# Autodesk Inventor assembly: sus1
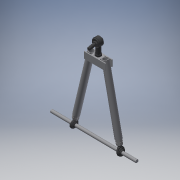
[picture p0: Inventor's stored thumbnail of the model, 180x180]
Saved by Autodesk Inventor 2018 (Build 220112000, 112)
## iProperties
Created: 2017-09-08
Part Number: sus1
Material: 一般
Document SubType Name: Assembly
Designer: mura5
Author: mura5
## Documents named in this file (8)
- C:\Users\mura5\Documents\RBBR\cart\Sus1.iam
- C:\Users\mura5\Documents\RBBR\cart\Rod1.iam
- C:\Users\mura5\Documents\RBBR\cart\Plate1.ipt
- C:\Users\mura5\Documents\RBBR\cart\Plate2.ipt
- C:\Users\mura5\Documents\RBBR\cart\iko_POS_14EC\AIS2016\POS 14ECBall.ipt
- C:\Users\mura5\Documents\RBBR\cart\Shaft14mm.ipt
- C:\Users\mura5\Documents\RBBR\cart\iko_LHSA_14\AIS2016\LHSA 14 Body1.ipt
- C:\Users\mura5\Documents\RBBR\cart\iko_LHSA_14\AIS2016\LHSA 14 Body2.ipt
## Components (10 placed, 7 different names)
1. POS 14ECBall:1 — 回転:1, 円柱状:1, ボール:4, メイト:9
2. Rod1:1 [sub-assembly] — 正接:2, 角度:1, メイト:2, ボール:4, メイト:6, メイト:7, 正接:3
3. Rod1:2 [sub-assembly] — ボール:2, 正接:1, 角度:2, メイト:3, メイト:5, メイト:8, 正接:4
4. Plate1:1 — 正接:1, 正接:2, フラッシュ:1, フラッシュ:2, メイト:1, フラッシュ:4, 正接:3, 正接:4
5. Plate2:1 — フラッシュ:1, フラッシュ:2, メイト:1, 角度:1, 角度:2, メイト:2, メイト:3, フラッシュ:3, メイト:4, リジッド:1, メイト:5, メイト:6, メイト:7, メイト:8
6. POS 14ECBall:2 — ボール:2, 回転:1, 円柱状:2, メイト:9
7. Shaft14mm:1 — 円柱状:1, 円柱状:2
8. Plate1:2 — フラッシュ:3, メイト:4, フラッシュ:4
9. LHSA 14 Body1:1 — リジッド:1, ボール:3
10. LHSA 14 Body2:1 — ボール:3
## Relationships (26: Mate 9, Tangent 4, Flush 4, BallJoint 3, CylindricalJoint 2, Angle 2, RevoluteJoint 1, WeldJoint 1)
- ボール:2 [BallJoint]: Rod1:2 ↔ POS 14ECBall:2
- 回転:1 [RevoluteJoint] (200 mm): POS 14ECBall:1 ↔ POS 14ECBall:2
- 円柱状:1 [CylindricalJoint]: POS 14ECBall:1 ↔ Shaft14mm:1
- 円柱状:2 [CylindricalJoint]: POS 14ECBall:2 ↔ Shaft14mm:1
- 正接:1 [Tangent]: Rod1:2 ↔ Plate1:1
- 正接:2 [Tangent]: Rod1:1 ↔ Plate1:1
- フラッシュ:1 [Flush] (-30 mm): Plate1:1 ↔ Plate2:1
- フラッシュ:2 [Flush]: Plate1:1 ↔ Plate2:1
- メイト:1 [Mate]: Plate1:1 ↔ Plate2:1
- 角度:1 [Angle] (-110 deg): Rod1:1 ↔ Plate2:1
- 角度:2 [Angle] (110 deg): Rod1:2 ↔ Plate2:1
- メイト:2 [Mate]: Rod1:1 ↔ Plate2:1
- メイト:3 [Mate]: Rod1:2 ↔ Plate2:1
- フラッシュ:3 [Flush]: Plate2:1 ↔ Plate1:2
- メイト:4 [Mate]: Plate2:1 ↔ Plate1:2
- フラッシュ:4 [Flush]: Plate1:1 ↔ Plate1:2
- リジッド:1 [WeldJoint]: Plate2:1 ↔ LHSA 14 Body1:1
- ボール:3 [BallJoint]: LHSA 14 Body1:1 ↔ LHSA 14 Body2:1
- ボール:4 [BallJoint]: POS 14ECBall:1 ↔ Rod1:1
- メイト:5 [Mate]: Rod1:2 ↔ Plate2:1
- メイト:6 [Mate]: Rod1:1 ↔ Plate2:1
- メイト:7 [Mate]: Rod1:1 ↔ Plate2:1
- メイト:8 [Mate]: Rod1:2 ↔ Plate2:1
- 正接:3 [Tangent]: Rod1:1 ↔ Plate1:1
- 正接:4 [Tangent]: Rod1:2 ↔ Plate1:1
- メイト:9 [Mate] (200 mm): POS 14ECBall:1 ↔ POS 14ECBall:2
